# Autodesk Inventor assembly: Assembly
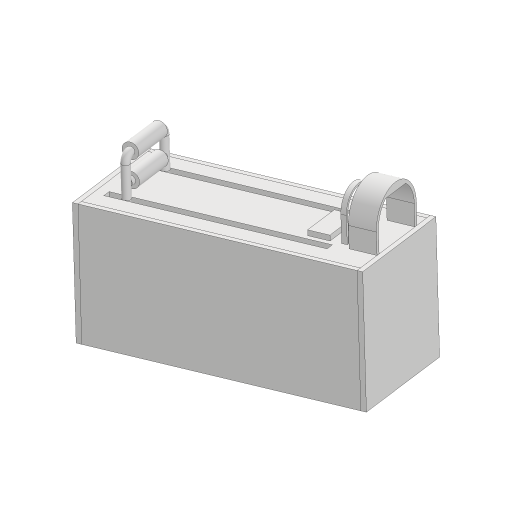
[picture p0: Inventor's stored thumbnail of the model, 512x512]
Saved by Autodesk Inventor 2023 (Build 270158000, 158)
## iProperties
Created: 2023-03-04
Part Number: Assembly
Document SubType Name: Assembly
Designer: Ethan Ko
Author: Ethan Ko
## Documents named in this file (15)
- C:\Users\Ethan Ko\Desktop\1P10\Team 29 DP3 CAD Parts\Assembly.iam
- C:\Users\Ethan Ko\Desktop\1P10\Team 29 DP3 CAD Parts\Ethan DP3 Parts\team29_box1(1).ipt
- C:\Users\Ethan Ko\Desktop\1P10\Team 29 DP3 CAD Parts\Ethan DP3 Parts\team29_box(2).ipt
- C:\Users\Ethan Ko\Desktop\1P10\Team 29 DP3 CAD Parts\Ethan DP3 Parts\team29_box(1).ipt
- C:\Users\Ethan Ko\Desktop\1P10\Team 29 DP3 CAD Parts\Ethan DP3 Parts\team29_gear_rod.ipt
- C:\Users\Ethan Ko\Desktop\1P10\Team 29 DP3 CAD Parts\Ethan DP3 Parts\team29_gear(2).ipt
- C:\Users\Ethan Ko\Desktop\1P10\Team 29 DP3 CAD Parts\Fariha DP3 Parts\Team29_BoxLid.ipt
- C:\Users\Ethan Ko\Desktop\1P10\Team 29 DP3 CAD Parts\Ethan DP3 Parts\team29_roller_attachment_final.ipt
- C:\Users\Ethan Ko\Desktop\1P10\Team 29 DP3 CAD Parts\Fariha DP3 Parts\Team29_Roller.ipt
- C:\Users\Ethan Ko\Desktop\1P10\Team 29 DP3 CAD Parts\Ethan DP3 Parts\team29_gear_attachment.ipt
- C:\Users\Ethan Ko\Desktop\1P10\Team 29 DP3 CAD Parts\Fariha DP3 Parts\Team29_SensorHolder.ipt
- C:\Users\Ethan Ko\Desktop\1P10\Team 29 DP3 CAD Parts\Fariha DP3 Parts\Team29_TubeHolder.ipt
- C:\Users\Ethan Ko\Desktop\1P10\Team 29 DP3 CAD Parts\Ethan DP3 Parts\team29_wall.ipt
- C:\Users\Ethan Ko\Desktop\1P10\Team 29 DP3 CAD Parts\Ethan DP3 Parts\team29_model_motor.ipt
- C:\Users\Ethan Ko\Desktop\1P10\Team 29 DP3 CAD Parts\Ethan DP3 Parts\team29_toothpaste_lift.ipt
## Components (44 placed, 14 different names)
1. team29_box1(1):1 — Mate:3, Flush:1, Flush:2, Mate:5, Mate:8, Mate:10, Mate:17, Mate:21, Mate:23, Mate:26, Mate:29, Mate:73, Mate:76, Mate:79, Mate:82, Mate:85, Mate:88, Mate:91, Mate:95, Mate:106
2. team29_box(1):1 — Mate:3, Flush:1, Flush:2, Flush:7, Flush:8, Mate:6, Mate:9, Mate:16, Mate:19, Mate:22, Mate:25, Mate:28, Mate:42
3. team29_box(2):2 — Mate:5, Flush:7, Flush:8, Mate:7, Mate:15, Mate:18, Mate:20, Mate:24, Mate:27, Mate:30, Flush:22, Mate:72, Mate:74, Mate:77, Mate:80, Mate:83, Mate:86, Mate:89, Mate:92, Mate:94
4. team29_gear_rod:1 — Mate:6, Mate:7, Mate:8, Mate:58, Flush:10, Mate:71
5. team29_gear_rod:2 — Mate:16, Mate:17, Mate:18, Mate:62, Flush:14
6. team29_gear_rod:3 — Mate:19, Mate:20, Mate:21, Mate:64, Flush:16
7. team29_gear_rod:4 — Mate:9, Mate:10, Mate:15, Mate:60, Flush:12
8. team29_gear_rod:5 — Mate:28, Mate:29, Mate:30, Mate:63, Flush:15
9. team29_gear_rod:6 — Mate:25, Mate:26, Mate:27, Mate:61, Flush:13
10. team29_gear_rod:7 — Mate:22, Mate:23, Mate:24, Mate:59, Flush:11
11. team29_gear(2):1 — Mate:62, Flush:14, Rotation:4, Rotation:5
12. team29_gear(2):2 — Mate:63, Flush:15, Rotation:5, Rotation:6
13. team29_gear(2):3 — Mate:61, Flush:13, Rotation:3, Rotation:4
14. team29_gear(2):4 — Mate:59, Flush:11, Rotation:1, Rotation:2
15. team29_gear(2):5 — Mate:60, Flush:12, Rotation:2, Rotation:3
16. team29_gear(2):6 — Mate:64, Flush:16, Rotation:6
17. team29_gear(2):7 — Mate:58, Flush:10, Rotation:1, Rotation/Translation:1, Mate:70, Rotation:13
18. Team29_BoxLid:1 — Mate:42, Mate:43, Mate:44, Mate:45, Mate:46, Mate:48, Mate:68, Mate:69, Flush:21, Flush:22, Mate:72, Flush:24, Mate:104, Flush:32, Mate:105, Flush:33, Flush:36
19. team29_roller_attachment_final:1 — Mate:44, Mate:48, Mate:49, Mate:51, Mate:56, Mate:57, Angle:2
20. team29_roller_attachment_final:2 — Mate:43, Mate:45, Mate:46, Mate:47, Mate:50, Mate:52, Mate:53, Mate:54, Mate:55, Angle:1
21. Team29_Roller:1 — Mate:47, Mate:49, Mate:50
22. Team29_Roller:2 — Mate:51, Mate:52, Mate:53
23. team29_gear_attachment:1 — Mate:56, Mate:57, Angle:2, Rotation/Translation:1
24. team29_gear_attachment:2 — Mate:54, Mate:55, Angle:1, Rotation/Translation:2
25. Team29_TubeHolder:1 — Mate:68, Mate:69, Flush:21
26. team29_wall:1 — Mate:73, Mate:74, Flush:24, Mate:75, Mate:78, Mate:81, Mate:84, Mate:87, Mate:90, Mate:93, Flush:31, Flush:34, Flush:35
27. team29_model_motor:1 — Mate:70, Mate:71, Mate:97, Rotation:13
28. team29_gear_rod:8 — Mate:90, Mate:91, Mate:92, Mate:102, Flush:29
29. team29_gear_rod:9 — Mate:93, Mate:94, Mate:95, Mate:103, Flush:30
30. team29_gear_rod:10 — Mate:87, Mate:88, Mate:89, Mate:101, Flush:28
31. team29_gear_rod:11 — Mate:75, Mate:76, Mate:77, Mate:96
32. team29_gear_rod:12 — Mate:84, Mate:85, Mate:86, Mate:100, Flush:27
33. team29_gear_rod:13 — Mate:81, Mate:82, Mate:83, Mate:99, Flush:26
34. team29_gear_rod:14 — Mate:78, Mate:79, Mate:80, Mate:98, Flush:25
35. team29_gear(2):8 — Mate:98, Flush:25, Rotation:8, Rotation:9
36. team29_gear(2):9 — Mate:99, Flush:26, Rotation:10, Rotation:11
37. team29_gear(2):10 — Mate:100, Flush:27, Rotation:12
38. team29_gear(2):11 — Mate:96, Mate:97, Rotation:7, Rotation/Translation:2
39. team29_gear(2):12 — Mate:102, Flush:29, Rotation:9, Rotation:10
40. team29_gear(2):13 — Mate:101, Flush:28, Rotation:7, Rotation:8
41. team29_gear(2):14 — Mate:103, Flush:30, Rotation:11, Rotation:12
42. Team29_SensorHolder:1 — Mate:104, Flush:31, Flush:32
43. team29_toothpaste_lift:1 — Mate:105, Flush:33, Flush:34
44. team29_box(2):3 — Mate:106, Flush:35, Flush:36
## Relationships (128: Mate 85, Flush 26, RelateRotation 13, Angle 2, RelateRotateTranslate 2)
- Mate:3: team29_box1(1):1 ↔ team29_box(1):1
- Flush:1: team29_box1(1):1 ↔ team29_box(1):1
- Flush:2: team29_box1(1):1 ↔ team29_box(1):1
- Mate:5: team29_box1(1):1 ↔ team29_box(2):2
- Flush:7: team29_box(1):1 ↔ team29_box(2):2
- Flush:8: team29_box(1):1 ↔ team29_box(2):2
- Mate:6: team29_box(1):1 ↔ team29_gear_rod:1
- Mate:7 (58 mm): team29_box(2):2 ↔ team29_gear_rod:1
- Mate:8 (65 mm): team29_box1(1):1 ↔ team29_gear_rod:1
- Mate:9: team29_box(1):1 ↔ team29_gear_rod:4
- Mate:10 (65 mm): team29_box1(1):1 ↔ team29_gear_rod:4
- Mate:15 (96 mm): team29_box(2):2 ↔ team29_gear_rod:4
- Mate:16: team29_box(1):1 ↔ team29_gear_rod:2
- Mate:17 (65 mm): team29_box1(1):1 ↔ team29_gear_rod:2
- Mate:18 (134 mm): team29_box(2):2 ↔ team29_gear_rod:2
- Mate:19: team29_box(1):1 ↔ team29_gear_rod:3
- Mate:20 (172 mm): team29_box(2):2 ↔ team29_gear_rod:3
- Mate:21 (65 mm): team29_box1(1):1 ↔ team29_gear_rod:3
- Mate:22: team29_box(1):1 ↔ team29_gear_rod:7
- Mate:23 (45 mm): team29_box1(1):1 ↔ team29_gear_rod:7
- Mate:24 (77 mm): team29_box(2):2 ↔ team29_gear_rod:7
- Mate:25: team29_box(1):1 ↔ team29_gear_rod:6
- Mate:26 (45 mm): team29_box1(1):1 ↔ team29_gear_rod:6
- Mate:27 (115 mm): team29_box(2):2 ↔ team29_gear_rod:6
- Mate:28: team29_box(1):1 ↔ team29_gear_rod:5
- Mate:29 (45 mm): team29_box1(1):1 ↔ team29_gear_rod:5
- Mate:30 (153 mm): team29_box(2):2 ↔ team29_gear_rod:5
- Mate:42: team29_box(1):1 ↔ Team29_BoxLid:1
- Mate:43: Team29_BoxLid:1 ↔ team29_roller_attachment_final:2
- Mate:44: Team29_BoxLid:1 ↔ team29_roller_attachment_final:1
- Mate:45: Team29_BoxLid:1 ↔ team29_roller_attachment_final:2
- Mate:46 (4 mm): Team29_BoxLid:1 ↔ team29_roller_attachment_final:2
- Mate:47: team29_roller_attachment_final:2 ↔ Team29_Roller:1
- Mate:48 (4 mm): Team29_BoxLid:1 ↔ team29_roller_attachment_final:1
- Mate:49: team29_roller_attachment_final:1 ↔ Team29_Roller:1
- Mate:50: team29_roller_attachment_final:2 ↔ Team29_Roller:1
- Mate:51: team29_roller_attachment_final:1 ↔ Team29_Roller:2
- Mate:52: team29_roller_attachment_final:2 ↔ Team29_Roller:2
- Mate:53: team29_roller_attachment_final:2 ↔ Team29_Roller:2
- Mate:54: team29_roller_attachment_final:2 ↔ team29_gear_attachment:2
- Mate:55: team29_roller_attachment_final:2 ↔ team29_gear_attachment:2
- Angle:1 (0 deg): team29_roller_attachment_final:2 ↔ team29_gear_attachment:2
- Mate:56: team29_roller_attachment_final:1 ↔ team29_gear_attachment:1
- Mate:57: team29_roller_attachment_final:1 ↔ team29_gear_attachment:1
- Angle:2 (0 deg): team29_roller_attachment_final:1 ↔ team29_gear_attachment:1
- Mate:58: team29_gear_rod:1 ↔ team29_gear(2):7
- Flush:10 (10 mm): team29_gear_rod:1 ↔ team29_gear(2):7
- Mate:59: team29_gear_rod:7 ↔ team29_gear(2):4
- Flush:11 (10 mm): team29_gear_rod:7 ↔ team29_gear(2):4
- Mate:60: team29_gear_rod:4 ↔ team29_gear(2):5
- Flush:12 (10 mm): team29_gear_rod:4 ↔ team29_gear(2):5
- Mate:61: team29_gear_rod:6 ↔ team29_gear(2):3
- Flush:13 (10 mm): team29_gear_rod:6 ↔ team29_gear(2):3
- Mate:62: team29_gear_rod:2 ↔ team29_gear(2):1
- Flush:14 (10 mm): team29_gear_rod:2 ↔ team29_gear(2):1
- Mate:63: team29_gear_rod:5 ↔ team29_gear(2):2
- Flush:15 (10 mm): team29_gear_rod:5 ↔ team29_gear(2):2
- Mate:64: team29_gear_rod:3 ↔ team29_gear(2):6
- Flush:16 (10 mm): team29_gear_rod:3 ↔ team29_gear(2):6
- Rotation:1 [RelateRotation] (1 ul): team29_gear(2):4 ↔ team29_gear(2):7
- Rotation:2 [RelateRotation] (1 ul): team29_gear(2):4 ↔ team29_gear(2):5
- Rotation:3 [RelateRotation] (1 ul): team29_gear(2):3 ↔ team29_gear(2):5
- Rotation:4 [RelateRotation] (1 ul): team29_gear(2):1 ↔ team29_gear(2):3
- Rotation:5 [RelateRotation] (1 ul): team29_gear(2):1 ↔ team29_gear(2):2
- Rotation:6 [RelateRotation] (1 ul): team29_gear(2):2 ↔ team29_gear(2):6
- Mate:68: Team29_BoxLid:1 ↔ Team29_TubeHolder:1
- Mate:69: Team29_BoxLid:1 ↔ Team29_TubeHolder:1
- Flush:21: Team29_BoxLid:1 ↔ Team29_TubeHolder:1
- Rotation/Translation:1 [RelateRotateTranslate] (30 mm): team29_gear(2):7 ↔ team29_gear_attachment:1
- Mate:70: team29_gear(2):7 ↔ team29_model_motor:1
- Mate:71: team29_gear_rod:1 ↔ team29_model_motor:1
- Flush:22: team29_box(2):2 ↔ Team29_BoxLid:1
- Mate:72: team29_box(2):2 ↔ Team29_BoxLid:1
- Mate:73: team29_box1(1):1 ↔ team29_wall:1
- Mate:74: team29_box(2):2 ↔ team29_wall:1
- Flush:24: Team29_BoxLid:1 ↔ team29_wall:1
- Mate:75: team29_wall:1 ↔ team29_gear_rod:11
- Mate:76 (65 mm): team29_box1(1):1 ↔ team29_gear_rod:11
- Mate:77 (58 mm): team29_box(2):2 ↔ team29_gear_rod:11
- Mate:78: team29_wall:1 ↔ team29_gear_rod:14
- Mate:79 (64 mm): team29_box1(1):1 ↔ team29_gear_rod:14
- Mate:80 (96 mm): team29_box(2):2 ↔ team29_gear_rod:14
- Mate:81: team29_wall:1 ↔ team29_gear_rod:13
- Mate:82 (65 mm): team29_box1(1):1 ↔ team29_gear_rod:13
- Mate:83 (134 mm): team29_box(2):2 ↔ team29_gear_rod:13
- Mate:84: team29_wall:1 ↔ team29_gear_rod:12
- Mate:85 (65 mm): team29_box1(1):1 ↔ team29_gear_rod:12
- Mate:86 (172 mm): team29_box(2):2 ↔ team29_gear_rod:12
- Mate:87: team29_wall:1 ↔ team29_gear_rod:10
- Mate:88 (45 mm): team29_box1(1):1 ↔ team29_gear_rod:10
- Mate:89 (77 mm): team29_box(2):2 ↔ team29_gear_rod:10
- Mate:90: team29_wall:1 ↔ team29_gear_rod:8
- Mate:91 (45 mm): team29_box1(1):1 ↔ team29_gear_rod:8
- Mate:92 (115 mm): team29_box(2):2 ↔ team29_gear_rod:8
- Mate:93: team29_wall:1 ↔ team29_gear_rod:9
- Mate:94 (153 mm): team29_box(2):2 ↔ team29_gear_rod:9
- Mate:95 (45 mm): team29_box1(1):1 ↔ team29_gear_rod:9
- Mate:96: team29_gear_rod:11 ↔ team29_gear(2):11
- Mate:97: team29_model_motor:1 ↔ team29_gear(2):11
- Mate:98: team29_gear_rod:14 ↔ team29_gear(2):8
- Flush:25 (-10 mm): team29_gear_rod:14 ↔ team29_gear(2):8
- Mate:99: team29_gear_rod:13 ↔ team29_gear(2):9
- Flush:26 (10 mm): team29_gear_rod:13 ↔ team29_gear(2):9
- Mate:100: team29_gear_rod:12 ↔ team29_gear(2):10
- Flush:27 (10 mm): team29_gear_rod:12 ↔ team29_gear(2):10
- Mate:101: team29_gear_rod:10 ↔ team29_gear(2):13
- Flush:28 (10 mm): team29_gear_rod:10 ↔ team29_gear(2):13
- Mate:102: team29_gear_rod:8 ↔ team29_gear(2):12
- Flush:29 (-10 mm): team29_gear_rod:8 ↔ team29_gear(2):12
- Mate:103: team29_gear_rod:9 ↔ team29_gear(2):14
- Flush:30 (-10 mm): team29_gear_rod:9 ↔ team29_gear(2):14
- Rotation:7 [RelateRotation] (1 ul): team29_gear(2):11 ↔ team29_gear(2):13
- Rotation:8 [RelateRotation] (1 ul): team29_gear(2):8 ↔ team29_gear(2):13
- Rotation:9 [RelateRotation] (1 ul): team29_gear(2):8 ↔ team29_gear(2):12
- Rotation:10 [RelateRotation] (1 ul): team29_gear(2):9 ↔ team29_gear(2):12
- Rotation:11 [RelateRotation] (1 ul): team29_gear(2):9 ↔ team29_gear(2):14
- Rotation:12 [RelateRotation] (1 ul): team29_gear(2):10 ↔ team29_gear(2):14
- Rotation/Translation:2 [RelateRotateTranslate] (94.2 mm): team29_gear_attachment:2 ↔ team29_gear(2):11
- Rotation:13 [RelateRotation] (1 ul): team29_gear(2):7 ↔ team29_model_motor:1
- Mate:104: Team29_BoxLid:1 ↔ Team29_SensorHolder:1
- Flush:31 (50 mm): team29_wall:1 ↔ Team29_SensorHolder:1
- Flush:32: Team29_BoxLid:1 ↔ Team29_SensorHolder:1
- Mate:105: Team29_BoxLid:1 ↔ team29_toothpaste_lift:1
- Flush:33 (45 mm): Team29_BoxLid:1 ↔ team29_toothpaste_lift:1
- Flush:34 (-35 mm): team29_wall:1 ↔ team29_toothpaste_lift:1
- Mate:106: team29_box1(1):1 ↔ team29_box(2):3
- Flush:35: team29_wall:1 ↔ team29_box(2):3
- Flush:36: Team29_BoxLid:1 ↔ team29_box(2):3
